# Autodesk Inventor assembly: Steering Assembly
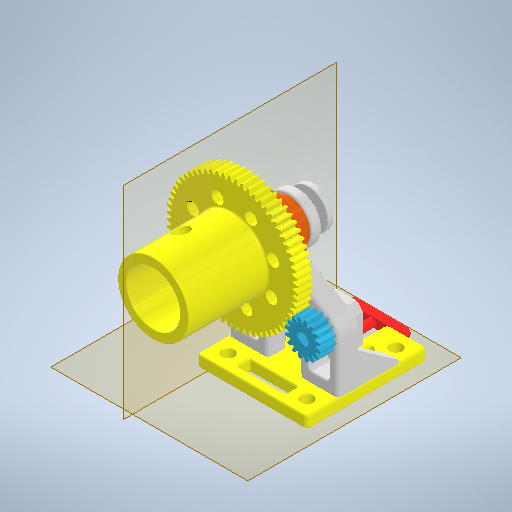
[picture p0: Inventor's stored thumbnail of the model, 512x512]
Saved by Autodesk Inventor 2025.2 (Build 292293000, 293)
## iProperties
Created: 2025-02-05
Part Number: Steering Assembly
Document SubType Name: Assembly
Designer: eason
Author: eason
## Documents named in this file (9)
- C:\Users\eason\Desktop\Code\Unojoy-Simulator-Rig\CAD\Steering\Steering Assembly.iam
- C:\Users\eason\Desktop\Code\Unojoy-Simulator-Rig\CAD\Steering\Steering Gear.ipt
- C:\Users\eason\Desktop\Code\Unojoy-Simulator-Rig\CAD\Steering\Encoder Gear.ipt
- C:\Users\eason\Desktop\Code\Unojoy-Simulator-Rig\CAD\Steering\Steering Gear Plate.ipt
- C:\Users\eason\Desktop\Code\Unojoy-Simulator-Rig\CAD\Steering\Steering Gear Plate 2.ipt
- C:\Users\eason\Desktop\Code\Unojoy-Simulator-Rig\CAD\Steering\Axle.ipt
- C:\Users\eason\Desktop\Code\Unojoy-Simulator-Rig\CAD\Steering\Steering Mounting Plate 1.ipt
- C:\Users\eason\Desktop\Code\Unojoy-Simulator-Rig\CAD\Steering\Steering Mounting Plate 2.ipt
- C:\Users\eason\Desktop\Code\Unojoy-Simulator-Rig\CAD\Steering\Steering Mounting Plate 3.ipt
## Components (8 placed, 8 different names)
1. Spur Gear1:1 — Insert:9
2. Spur Gear2:1 — Angle:2, Insert:8
3. Steering Gear Plate:1 — Insert:2, Angle:1, Insert:3, Insert:4
4. Steering Gear Plate 2:1 — Insert:3, Insert:4
5. Steering Mounting Plate 1:1 — Mate:18, Mate:20, Insert:7, Insert:9, Mate:21
6. Steering Mounting Plate 2:1 — Mate:17, Mate:18, Mate:19, Mate:20, Flush:1, Insert:5, Insert:6, Mate:21
7. Axle:1 — Insert:2, Angle:1, Insert:7, Angle:2, Insert:8
8. Steering Mounting Plate 3:1 — Insert:5, Insert:6
## Relationships (16: Insert 8, Mate 5, Angle 2, Flush 1)
- Mate:17: Steering Mounting Plate 2:1
- Mate:18: Steering Mounting Plate 1:1 ↔ Steering Mounting Plate 2:1
- Mate:19: Steering Mounting Plate 2:1
- Mate:20: Steering Mounting Plate 1:1 ↔ Steering Mounting Plate 2:1
- Flush:1: Steering Mounting Plate 2:1
- Insert:2 (-5.2 mm): Steering Gear Plate:1 ↔ Axle:1
- Angle:1 (0 deg): Steering Gear Plate:1 ↔ Axle:1
- Insert:3: Steering Gear Plate:1 ↔ Steering Gear Plate 2:1
- Insert:4: Steering Gear Plate:1 ↔ Steering Gear Plate 2:1
- Insert:5: Steering Mounting Plate 2:1 ↔ Steering Mounting Plate 3:1
- Insert:6: Steering Mounting Plate 2:1 ↔ Steering Mounting Plate 3:1
- Insert:7 (-0.1 mm): Steering Mounting Plate 1:1 ↔ Axle:1
- Angle:2 (0 deg): Spur Gear2:1 ↔ Axle:1
- Insert:8 (9 mm): Spur Gear2:1 ↔ Axle:1
- Insert:9: Spur Gear1:1 ↔ Steering Mounting Plate 1:1
- Mate:21: Steering Mounting Plate 1:1 ↔ Steering Mounting Plate 2:1
